# Autodesk Inventor assembly: Assembly
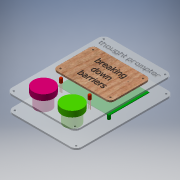
[picture p0: Inventor's stored thumbnail of the model, 180x180]
Saved by Autodesk Inventor 2016 (Build 200138000, 138)
## iProperties
Created: 2015-09-18
Part Number: Assembly
Document SubType Name: Assembly
Designer: Erin
Author: Erin
## Documents named in this file (8)
- C:\Users\Erin\Desktop\STEAMLabs\Assembly.iam
- C:\Users\Erin\Desktop\STEAMLabs\protoboard.ipt
- C:\Users\Erin\Desktop\STEAMLabs\arduinopromini.ipt
- C:\Users\Erin\Desktop\STEAMLabs\button.ipt
- C:\Users\Erin\Desktop\STEAMLabs\5mm_led.ipt
- C:\Users\Erin\Desktop\STEAMLabs\FrontPanel.ipt
- C:\Users\Erin\Desktop\STEAMLabs\BackPanel.ipt
- C:\Users\Erin\Desktop\STEAMLabs\PromptPanel.ipt
## Components (9 placed, 7 different names)
1. arduinopromini:1
2. 5mm_led:1 — Insert:4
3. 5mm_led:2 — Insert:3
4. button:1 — Insert:1
5. button:2 — Insert:2
6. FrontPanel:1 — Insert:1, Insert:2, Insert:3, Insert:4, Insert:5
7. BackPanel:1
8. PromptPanel:1 — Insert:5
9. protoboard:2
## Relationships (5: Insert 5)
- Insert:1: button:1 ↔ FrontPanel:1
- Insert:2: button:2 ↔ FrontPanel:1
- Insert:3: 5mm_led:2 ↔ FrontPanel:1
- Insert:4: 5mm_led:1 ↔ FrontPanel:1
- Insert:5: FrontPanel:1 ↔ PromptPanel:1
